# Autodesk Inventor assembly: Assembly
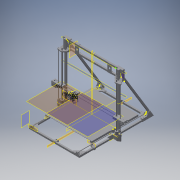
[picture p0: Inventor's stored thumbnail of the model, 180x180]
Saved by Autodesk Inventor 2016 (Build 200138000, 138)
## iProperties
Created: 2016-05-26
Part Number: Assembly
Document SubType Name: Assembly
Designer: Scott
Author: Scott
## Documents named in this file (36)
- C:\Users\Scott\Google Drive\Engineering Ideas and Designs\3D printer\Dynamo Printer\Parts\Rebuild\Assembly.iam
- C:\Users\Scott\Google Drive\Engineering Ideas and Designs\3D printer\Dynamo Printer\Parts\Rebuild\Alum extrusion 26in.ipt
- C:\Users\Scott\Google Drive\Engineering Ideas and Designs\3D printer\Dynamo Printer\Parts\Rebuild\Alum extrusion 39_5in.ipt
- C:\Users\Scott\Google Drive\Engineering Ideas and Designs\3D printer\Dynamo Printer\Parts\Rebuild\Bed Bracket.ipt
- C:\Users\Scott\Google Drive\Engineering Ideas and Designs\3D printer\Dynamo Printer\Parts\Rebuild\Bed Bracket_MIR.ipt
- C:\Users\Scott\Google Drive\Engineering Ideas and Designs\3D printer\Dynamo Printer\Parts\Rebuild\Be Rails.ipt
- C:\Users\Scott\Google Drive\Engineering Ideas and Designs\3D printer\Dynamo Printer\Parts\Rebuild\Alum Bed plate.ipt
- C:\Users\Scott\Google Drive\Engineering Ideas and Designs\3D printer\Dynamo Printer\Parts\Rebuild\verticle connnector.ipt
- C:\Users\Scott\Google Drive\Engineering Ideas and Designs\3D printer\Dynamo Printer\Parts\Rebuild\MotorandLeadscrew.ipt
- C:\Users\Scott\Google Drive\Engineering Ideas and Designs\3D printer\Dynamo Printer\Parts\Rebuild\MotorandLeadscrew_MIR.ipt
- C:\Users\Scott\Google Drive\Engineering Ideas and Designs\3D printer\Dynamo Printer\Parts\Rebuild\Alum extrusion 30in.ipt
- C:\Users\Scott\Google Drive\Engineering Ideas and Designs\3D printer\Dynamo Printer\Parts\Rebuild\Z rails.ipt
- C:\Users\Scott\Google Drive\Engineering Ideas and Designs\3D printer\Dynamo Printer\Parts\Rebuild\verticle connnector_MIR.ipt
- C:\Users\Scott\Google Drive\Engineering Ideas and Designs\3D printer\Dynamo Printer\Parts\Rebuild\Alum extrusion 30in_MIR.ipt
- C:\Users\Scott\Google Drive\Engineering Ideas and Designs\3D printer\Dynamo Printer\Parts\Rebuild\Z rails_MIR.ipt
- C:\Users\Scott\Google Drive\Engineering Ideas and Designs\3D printer\Dynamo Printer\Parts\Rebuild\Z Upper End.ipt
- C:\Users\Scott\Google Drive\Engineering Ideas and Designs\3D printer\Dynamo Printer\Parts\Rebuild\Z Upper End_MIR.ipt
- C:\Users\Scott\Google Drive\Engineering Ideas and Designs\3D printer\Dynamo Printer\Parts\Rebuild\BracerBedMountpoint.ipt
- C:\Users\Scott\Google Drive\Engineering Ideas and Designs\3D printer\Dynamo Printer\Parts\Rebuild\BracerBedMountpoint_MIR.ipt
- C:\Users\Scott\Google Drive\Engineering Ideas and Designs\3D printer\Dynamo Printer\Parts\Rebuild\Alum 32in bar.ipt
- C:\Users\Scott\Google Drive\Engineering Ideas and Designs\3D printer\Dynamo Printer\Parts\Rebuild\Alum 32in bar_MIR.ipt
- C:\Users\Scott\Google Drive\Engineering Ideas and Designs\3D printer\Dynamo Printer\Parts\Rebuild\Xendmotorside.ipt
- C:\Users\Scott\Google Drive\Engineering Ideas and Designs\3D printer\Dynamo Printer\Parts\Rebuild\Xrails.ipt
- C:\Users\Scott\Google Drive\Engineering Ideas and Designs\3D printer\Dynamo Printer\Parts\Rebuild\ExtruderMount.ipt
- C:\Users\Scott\Google Drive\Engineering Ideas and Designs\3D printer\Dynamo Printer\Parts\Rebuild\XendmotorsideIdler.ipt
- C:\Users\Scott\Google Drive\Engineering Ideas and Designs\3D printer\Dynamo Printer\Parts\Rebuild\X Carriage.ipt
- C:\Users\Scott\Google Drive\Engineering Ideas and Designs\3D printer\Dynamo Printer\Parts\Rebuild\SecondExtruder.ipt
- C:\Users\Scott\Google Drive\Engineering Ideas and Designs\3D printer\Dynamo Printer\Parts\Rebuild\Bed Slider.ipt
- C:\Users\Scott\Google Drive\Engineering Ideas and Designs\3D printer\Dynamo Printer\Parts\Rebuild\Bed SliderIdler.ipt
- C:\Users\Scott\Google Drive\Engineering Ideas and Designs\3D printer\Dynamo Printer\Parts\Rebuild\Ross Rail.ipt
- C:\Users\Scott\Google Drive\Engineering Ideas and Designs\3D printer\Dynamo Printer\Parts\Rebuild\YMotorMount.ipt
- C:\Users\Scott\Google Drive\Engineering Ideas and Designs\3D printer\Dynamo Printer\Parts\Rebuild\Y belt mount point.ipt
- C:\Users\Scott\Google Drive\Engineering Ideas and Designs\3D printer\Dynamo Printer\Parts\Rebuild\YIdler.ipt
- C:\Users\Scott\Google Drive\Engineering Ideas and Designs\3D printer\Dynamo Printer\Parts\Rebuild\Hotend mount.ipt
- C:\Users\Scott\Google Drive\Engineering Ideas and Designs\3D printer\Dynamo Printer\Parts\Rebuild\Braces.ipt
- C:\Users\Scott\Google Drive\Engineering Ideas and Designs\3D printer\Dynamo Printer\Parts\Rebuild\Extruder Holder and Fans.ipt
## Components (41 placed, 35 different names)
1. Alum extrusion 26in:1 — Mate:1, Mate:2, Mate:3, Mate:4, Mate:5, Mate:6, Flush:1, Flush:2, Symmetry:2, Flush:50
2. Alum extrusion 26in:2 — Mate:7, Mate:8, Mate:9, Mate:10, Mate:11, Mate:12, Symmetry:2, Mate:13
3. Alum extrusion 39_5in:1 — Mate:4, Mate:5, Mate:6, Mate:7, Mate:8, Symmetry:1, Mate:14, Flush:5
4. Alum extrusion 39_5in:2 — Mate:1, Mate:2, Mate:3, Mate:9, Symmetry:1, Flush:6, Flush:7
5. Bed Bracket:1 — Flush:1, Flush:2, Flush:3, Flush:4
6. Bed Bracket:2 — Mate:10, Mate:11, Mate:12, Flush:20, Flush:21, Mate:27, Mate:28, Flush:23
7. Bed Bracket_MIR:1 — Flush:51
8. Bed Bracket_MIR:2 — Mate:13, Mate:14
9. Be Rails:1 — Flush:3, Flush:4
10. Alum Bed plate:1 — Flush:39, Flush:40, Flush:41, Flush:42
11. verticle connnector:1 — Flush:5, Flush:6, Flush:8, Mate:15, Mate:16, Flush:9, Flush:10, Mate:17, Mate:18, Flush:11, Flush:12, Flush:13, Flush:14, Flush:15, Flush:16
12. MotorandLeadscrew:1 — Flush:7, Flush:8, Mate:15, Mate:16, Flush:9
13. MotorandLeadscrew_MIR:1 — Flush:27
14. Alum extrusion 30in:1 — Flush:10, Mate:17, Mate:18, Flush:15, Flush:16, Symmetry:3
15. Z rails:1 — Flush:11, Flush:12, Flush:13, Flush:14, Flush:18
16. verticle connnector_MIR:1 — Mate:19, Mate:20, Mate:21, Mate:22, Flush:17, Mate:23, Mate:24, Mate:25, Mate:26
17. Alum extrusion 30in_MIR:1 — Mate:19, Mate:20, Mate:21, Mate:22, Flush:17, Symmetry:3
18. Z rails_MIR:1 — Mate:23, Mate:24, Mate:25, Mate:26
19. Z Upper End:1 — Flush:18, Flush:19, Flush:22, Flush:24, Flush:25
20. Z Upper End_MIR:1 — Flush:32
21. Alum extrusion 30in:2 — Flush:26
22. Alum extrusion 30in:3 — Flush:19
23. BracerBedMountpoint:1 — Flush:20, Flush:21, Flush:22, Mate:27, Mate:28, Flush:23, Flush:24
24. BracerBedMountpoint_MIR:1
25. Alum 32in bar:1 — Flush:25
26. Alum 32in bar_MIR:1
27. Xendmotorside:1 — Flush:28, Flush:29, Flush:30, Flush:31, Flush:35
28. Xrails:1 — Flush:30, Flush:31
29. ExtruderMount:1 — Flush:33, Flush:34
30. XendmotorsideIdler:1 — Mate:29, Mate:30
31. X Carriage:1 — Flush:36, Flush:37, Flush:49
32. SecondExtruder:1 — Flush:38
33. Bed Slider:1 — Flush:39, Flush:40
34. Bed SliderIdler:1
35. Ross Rail:1 — Flush:41, Flush:42, Flush:45
36. YMotorMount:1 — Flush:43, Flush:44, Flush:46, Flush:48
37. Y belt mount point:1 — Flush:45, Flush:46, Flush:47
38. YIdler:1 — Flush:47, Flush:48
39. Hotend mount:1 — Flush:49, Flush:52, Flush:53
40. Braces:1 — Flush:50, Flush:51
41. Extruder Holder and Fans:1 — Flush:52, Flush:53
## Relationships (86: Flush 53, Mate 30, Symmetry 3)
- Mate:1: Alum extrusion 26in:1 ↔ Alum extrusion 39_5in:2
- Mate:2: Alum extrusion 26in:1 ↔ Alum extrusion 39_5in:2
- Mate:3: Alum extrusion 26in:1 ↔ Alum extrusion 39_5in:2
- Mate:4: Alum extrusion 26in:1 ↔ Alum extrusion 39_5in:1
- Mate:5: Alum extrusion 26in:1 ↔ Alum extrusion 39_5in:1
- Mate:6: Alum extrusion 26in:1 ↔ Alum extrusion 39_5in:1
- Mate:7: Alum extrusion 26in:2 ↔ Alum extrusion 39_5in:1
- Mate:8: Alum extrusion 26in:2 ↔ Alum extrusion 39_5in:1
- Mate:9: Alum extrusion 26in:2 ↔ Alum extrusion 39_5in:2
- Flush:1: Alum extrusion 26in:1 ↔ Bed Bracket:1
- Flush:2: Alum extrusion 26in:1 ↔ Bed Bracket:1
- Mate:10: Alum extrusion 26in:2 ↔ Bed Bracket:2
- Mate:11: Alum extrusion 26in:2 ↔ Bed Bracket:2
- Mate:12: Alum extrusion 26in:2 ↔ Bed Bracket:2
- Symmetry:1: Alum extrusion 39_5in:1 ↔ Alum extrusion 39_5in:2
- Symmetry:2: Alum extrusion 26in:1 ↔ Alum extrusion 26in:2
- Flush:3: Bed Bracket:1 ↔ Be Rails:1
- Flush:4: Bed Bracket:1 ↔ Be Rails:1
- Mate:13: Alum extrusion 26in:2 ↔ Bed Bracket_MIR:2
- Mate:14: Alum extrusion 39_5in:1 ↔ Bed Bracket_MIR:2
- Flush:5: Alum extrusion 39_5in:1 ↔ verticle connnector:1
- Flush:6: Alum extrusion 39_5in:2 ↔ verticle connnector:1
- Flush:7: Alum extrusion 39_5in:2 ↔ MotorandLeadscrew:1
- Flush:8: verticle connnector:1 ↔ MotorandLeadscrew:1
- Mate:15: verticle connnector:1 ↔ MotorandLeadscrew:1
- Mate:16: verticle connnector:1 ↔ MotorandLeadscrew:1
- Flush:9: verticle connnector:1 ↔ MotorandLeadscrew:1
- Flush:10: verticle connnector:1 ↔ Alum extrusion 30in:1
- Mate:17: verticle connnector:1 ↔ Alum extrusion 30in:1
- Mate:18: verticle connnector:1 ↔ Alum extrusion 30in:1
- Flush:11: verticle connnector:1 ↔ Z rails:1
- Flush:12: verticle connnector:1 ↔ Z rails:1
- Flush:13: verticle connnector:1 ↔ Z rails:1
- Flush:14: verticle connnector:1 ↔ Z rails:1
- Flush:15: verticle connnector:1 ↔ Alum extrusion 30in:1
- Flush:16: verticle connnector:1 ↔ Alum extrusion 30in:1
- Mate:19: verticle connnector_MIR:1 ↔ Alum extrusion 30in_MIR:1
- Mate:20: verticle connnector_MIR:1 ↔ Alum extrusion 30in_MIR:1
- Mate:21: verticle connnector_MIR:1 ↔ Alum extrusion 30in_MIR:1
- Mate:22: verticle connnector_MIR:1 ↔ Alum extrusion 30in_MIR:1
- Flush:17: verticle connnector_MIR:1 ↔ Alum extrusion 30in_MIR:1
- Mate:23: verticle connnector_MIR:1 ↔ Z rails_MIR:1
- Mate:24: verticle connnector_MIR:1 ↔ Z rails_MIR:1
- Mate:25: verticle connnector_MIR:1 ↔ Z rails_MIR:1
- Mate:26: verticle connnector_MIR:1 ↔ Z rails_MIR:1
- Flush:18: Z rails:1 ↔ Z Upper End:1
- Symmetry:3: Alum extrusion 30in:1 ↔ Alum extrusion 30in_MIR:1
- Flush:19: Z Upper End:1 ↔ Alum extrusion 30in:3
- Flush:20: Bed Bracket:2 ↔ BracerBedMountpoint:1
- Flush:21: Bed Bracket:2 ↔ BracerBedMountpoint:1
- Flush:22: Z Upper End:1 ↔ BracerBedMountpoint:1
- Mate:27: Bed Bracket:2 ↔ BracerBedMountpoint:1
- Mate:28: Bed Bracket:2 ↔ BracerBedMountpoint:1
- Flush:23: Bed Bracket:2 ↔ BracerBedMountpoint:1
- Flush:24: Z Upper End:1 ↔ BracerBedMountpoint:1
- Flush:25: Z Upper End:1 ↔ Alum 32in bar:1
- Flush:26 (174.625 mm): Alum extrusion 30in:2
- Flush:27 (166.6875 mm): MotorandLeadscrew_MIR:1
- Flush:28: Xendmotorside:1
- Flush:29: Xendmotorside:1
- Flush:30: Xendmotorside:1 ↔ Xrails:1
- Flush:31: Xendmotorside:1 ↔ Xrails:1
- Flush:32 (63.5 mm): Z Upper End_MIR:1
- Flush:33: ExtruderMount:1
- Flush:34: ExtruderMount:1
- Mate:29: XendmotorsideIdler:1
- Mate:30: XendmotorsideIdler:1
- Flush:35 (127 mm): Xendmotorside:1
- Flush:36: X Carriage:1
- Flush:37: X Carriage:1
- Flush:38: SecondExtruder:1
- Flush:39: Alum Bed plate:1 ↔ Bed Slider:1
- Flush:40 (-304.8 mm): Alum Bed plate:1 ↔ Bed Slider:1
- Flush:41: Alum Bed plate:1 ↔ Ross Rail:1
- Flush:42: Alum Bed plate:1 ↔ Ross Rail:1
- Flush:43: YMotorMount:1
- Flush:44: YMotorMount:1
- Flush:45: Ross Rail:1 ↔ Y belt mount point:1
- Flush:46: YMotorMount:1 ↔ Y belt mount point:1
- Flush:47: Y belt mount point:1 ↔ YIdler:1
- Flush:48: YMotorMount:1 ↔ YIdler:1
- Flush:49: X Carriage:1 ↔ Hotend mount:1
- Flush:50: Alum extrusion 26in:1 ↔ Braces:1
- Flush:51 (-207.9752 mm): Bed Bracket_MIR:1 ↔ Braces:1
- Flush:52: Hotend mount:1 ↔ Extruder Holder and Fans:1
- Flush:53: Hotend mount:1 ↔ Extruder Holder and Fans:1
